# Autodesk Inventor assembly: map #2
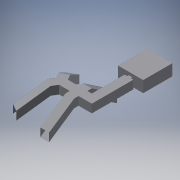
[picture p0: Inventor's stored thumbnail of the model, 180x180]
Saved by Autodesk Inventor 2017 (Build 210142000, 142)
## iProperties
Created: 2018-05-09
Part Number: map #2
Document SubType Name: Assembly
Designer: braxtonwright
Author: braxtonwright
## Documents named in this file (7)
- D:\School\Game develpment\geoscape\assembly\map #2.iam
- D:\School\Game develpment\geoscape\done\lowend map componts\corridors\corridor.ipt
- D:\School\Game develpment\geoscape\done\lowend map componts\corridors\corridor 90 turn.ipt
- D:\School\Game develpment\geoscape\done\lowend map componts\corridors\X corridor.ipt
- D:\School\Game develpment\geoscape\done\lowend map componts\corridors\Y corridor.ipt
- D:\School\Game develpment\geoscape\rooms\starting room.ipt
- D:\School\Game develpment\geoscape\corridors\ramp.ipt
## Components (18 placed, 6 different names)
1. corridor:1 — Flush:1, Flush:5, Mate:1, Mate:5, Mate:6
2. corridor:2 — Flush:1, Flush:2, Flush:5, Flush:6, Mate:1, Mate:2
3. corridor 90 turn:2 — Flush:2, Flush:3, Flush:6, Flush:7, Mate:2, Mate:3
4. X corridor:1 — Flush:3, Flush:4, Flush:7, Flush:8, Mate:3, Mate:4, Mate:7, Mate:10, Mate:19, Mate:22
5. Y corridor:1 — Flush:4, Flush:8, Mate:4, Mate:8, Mate:9, Mate:20, Mate:21
6. starting room:1 — Mate:5, Mate:6
7. ramp:1 — Mate:9, Flush:17, Mate:15, Mate:20
8. ramp:2 — Flush:19, Flush:20, Mate:17, Mate:18
9. ramp:3 — Flush:20, Mate:18
10. ramp:4 — Mate:10, Flush:19, Mate:17, Mate:19
11. ramp:5 — Flush:17, Flush:18, Mate:15, Mate:16
12. ramp:6 — Flush:18, Mate:16
13. ramp:7 — Mate:8, Flush:15, Mate:13, Mate:21
14. ramp:8 — Flush:15, Flush:16, Mate:13, Mate:14
15. ramp:9 — Flush:16, Mate:14
16. ramp:10 — Mate:7, Flush:13, Mate:11, Mate:22
17. ramp:11 — Flush:13, Flush:14, Mate:11, Mate:12
18. ramp:12 — Flush:14, Mate:12
## Relationships (38: Mate 22, Flush 16)
- Flush:1: corridor:1 ↔ corridor:2
- Flush:2: corridor:2 ↔ corridor 90 turn:2
- Flush:3: corridor 90 turn:2 ↔ X corridor:1
- Flush:4: X corridor:1 ↔ Y corridor:1
- Flush:5: corridor:1 ↔ corridor:2
- Flush:6: corridor:2 ↔ corridor 90 turn:2
- Flush:7: corridor 90 turn:2 ↔ X corridor:1
- Flush:8: X corridor:1 ↔ Y corridor:1
- Mate:1: corridor:1 ↔ corridor:2
- Mate:2: corridor:2 ↔ corridor 90 turn:2
- Mate:3: corridor 90 turn:2 ↔ X corridor:1
- Mate:4: X corridor:1 ↔ Y corridor:1
- Mate:5: corridor:1 ↔ starting room:1
- Mate:6: corridor:1 ↔ starting room:1
- Mate:7: X corridor:1 ↔ ramp:10
- Mate:8: Y corridor:1 ↔ ramp:7
- Mate:9: Y corridor:1 ↔ ramp:1
- Mate:10: X corridor:1 ↔ ramp:4
- Flush:13: ramp:10 ↔ ramp:11
- Flush:14: ramp:11 ↔ ramp:12
- Mate:11: ramp:10 ↔ ramp:11
- Mate:12: ramp:11 ↔ ramp:12
- Flush:15: ramp:7 ↔ ramp:8
- Flush:16: ramp:8 ↔ ramp:9
- Mate:13: ramp:7 ↔ ramp:8
- Mate:14: ramp:8 ↔ ramp:9
- Flush:17: ramp:1 ↔ ramp:5
- Flush:18: ramp:5 ↔ ramp:6
- Mate:15: ramp:1 ↔ ramp:5
- Mate:16: ramp:5 ↔ ramp:6
- Flush:19: ramp:2 ↔ ramp:4
- Flush:20: ramp:2 ↔ ramp:3
- Mate:17: ramp:2 ↔ ramp:4
- Mate:18: ramp:2 ↔ ramp:3
- Mate:19: X corridor:1 ↔ ramp:4
- Mate:20: Y corridor:1 ↔ ramp:1
- Mate:21: Y corridor:1 ↔ ramp:7
- Mate:22: X corridor:1 ↔ ramp:10
